# Autodesk Inventor assembly: ASSY_TREBUCHET_DESIGN2
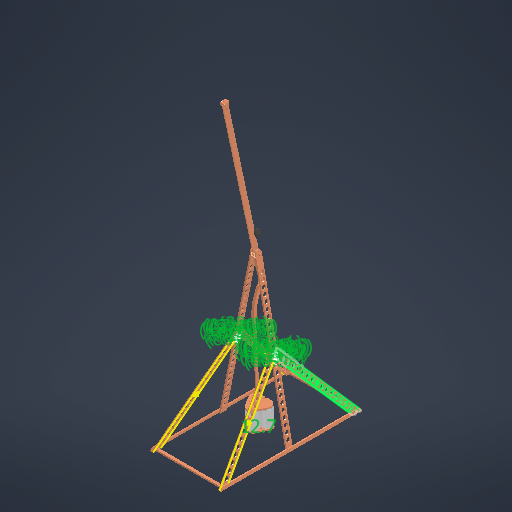
[picture p0: Inventor's stored thumbnail of the model, 512x512]
Saved by Autodesk Inventor 2026.2 (Build 302298010, 298A)
## iProperties
Created: 2026-02-10
Part Number: ASSY_TREBUCHET_DESIGN2
Document SubType Name: Assembly
Designer: 4aida
Mass: 1736.51 g
Surface Area: 8151.09 cm^2
Volume: 2284.88 cm^3
Density: 0.76 g/cm^3
Author: 4aida
## Documents named in this file (17)
- C:\Users\4aida\OneDrive\Documents\GitHub\Design_II_Group6\Trebuchet\WIPPER_TREBUCHET\ASSY_TREBUCHET_DESIGN2.iam
- C:\Users\4aida\OneDrive\Documents\GitHub\Design_II_Group6\Trebuchet\Canette-355ml.ipt
- C:\Users\4aida\OneDrive\Documents\GitHub\Design_II_Group6\Trebuchet\Yellow_dot_squash_ball,Trebuchet.ipt
- C:\Users\4aida\OneDrive\Documents\GitHub\Design_II_Group6\Trebuchet\WIPPER_TREBUCHET\wipper_arm.ipt
- C:\Users\4aida\OneDrive\Documents\GitHub\Design_II_Group6\Trebuchet\COUNTERWEIGHT_OUTSIDE_ARM,TREBUCHET.ipt
- C:\Users\4aida\OneDrive\Documents\GitHub\Design_II_Group6\Trebuchet\WIPPER_TREBUCHET\BASE_FRONT,BACK_TREBUCHET.ipt
- C:\Users\4aida\OneDrive\Documents\GitHub\Design_II_Group6\Trebuchet\WIPPER_TREBUCHET\BASE_SIDEK_TREBUCHET.ipt
- C:\Users\4aida\OneDrive\Documents\GitHub\Design_II_Group6\Trebuchet\WIPPER_TREBUCHET\UPRIGHTS_TREBUCHET.ipt
- C:\Users\4aida\OneDrive\Documents\GitHub\Design_II_Group6\Trebuchet\WIPPER_TREBUCHET\SUPPORTS_TREBUCHET.ipt
- C:\Users\4aida\OneDrive\Documents\GitHub\Design_II_Group6\Trebuchet\WIPPER_TREBUCHET\BOTTOM_PLATE_WEIGHTS_TREBUCHET.ipt
- C:\Users\4aida\OneDrive\Documents\GitHub\Design_II_Group6\Trebuchet\WIPPER_TREBUCHET\TRI_SPACER_TOP_TREBUCHET.ipt
- C:\Users\4aida\OneDrive\Documents\GitHub\Design_II_Group6\Trebuchet\WIPPER_TREBUCHET\MAIN_PIVOT_DOWEL_TREBUCHET.ipt
- C:\Users\4aida\OneDrive\Documents\GitHub\Design_II_Group6\Trebuchet\WIPPER_TREBUCHET\CW_PIVOT_TREBUCHET.ipt
- C:\Users\4aida\OneDrive\Documents\GitHub\Design_II_Group6\Trebuchet\WIPPER_TREBUCHET\TOP_PLATE_WEIGHTS_TREBUCHET.ipt
- C:\Users\4aida\OneDrive\Documents\GitHub\Design_II_Group6\Trebuchet\WIPPER_TREBUCHET\CONTERWEIGHT_SHAFT_TREBUCHET.ipt
- C:\Users\4aida\OneDrive\Documents\GitHub\Design_II_Group6\Trebuchet\WIPPER_TREBUCHET\RELEASE_BLOCK_TREBUCHET.ipt
- C:\Users\4aida\OneDrive\Documents\GitHub\Design_II_Group6\Trebuchet\WIPPER_TREBUCHET\RELEASE_BLOCK_PINS_TREBUCHET.ipt
## Components (27 placed, 16 different names)
1. Yellow_dot_squash_ball,Trebuchet:1 — Mate:45, Mate:85
2. BASE_FRONT,BACK_TREBUCHET:1 — Flush:40, Flush:42, Mate:94
3. BASE_FRONT,BACK_TREBUCHET:3 — Flush:28, Flush:41, Flush:42, Mate:95
4. UPRIGHTS_TREBUCHET:1 — Mate:38, Flush:29, Flush:30, Mate:48, Mate:49, Mate:50, Flush:39, Flush:41, Mate:60, Flush:44, Mate:61, Mate:64, Mate:89, Flush:56, Mate:90, Mate:92
5. UPRIGHTS_TREBUCHET:2 — Flush:31, Flush:32, Mate:46, Mate:47, Mate:50, Flush:39, Angle:1, Flush:40, Mate:58, Mate:59, Flush:43, Mate:88, Flush:54, Mate:91, Mate:93
6. wipper_arm:3 — Mate:39, Mate:44, Mate:45, Mate:55, Mate:56, Flush:45, Mate:66, Mate:75, Mate:76, Mate:77, Mate:78, Mate:79, Mate:82, Mate:85
7. SUPPORTS_TREBUCHET:1 — Flush:30, Mate:49, Mate:92, Mate:94
8. SUPPORTS_TREBUCHET:2 — Flush:32, Mate:46, Flush:53, Mate:91
9. SUPPORTS_TREBUCHET:3 — Flush:29, Mate:48, Flush:55, Mate:90, Mate:95
10. SUPPORTS_TREBUCHET:4 — Flush:31, Mate:47, Mate:93
11. COUNTERWEIGHT_OUTSIDE_ARM,TREBUCHET:3 — Mate:55, Mate:56, Mate:65, Mate:67, Mate:68, Mate:69, Insert:1
12. TRI_SPACER_TOP_TREBUCHET:1 — Mate:60, Flush:44, Mate:61, Mate:76
13. TRI_SPACER_TOP_TREBUCHET:2 — Mate:58, Mate:59, Flush:43, Mate:75
14. MAIN_PIVOT_DOWEL_TREBUCHET:1 — Mate:64, Flush:45
15. CW_PIVOT_TREBUCHET:1 — Mate:65, Mate:66
16. BOTTOM_PLATE_WEIGHTS_TREBUCHET:1 — Flush:48, Flush:49, Mate:74
17. TOP_PLATE_WEIGHTS_TREBUCHET:1 — Mate:67, Mate:68, Mate:69, Mate:70, Mate:71, Mate:72, Mate:73, Flush:48, Flush:49, Mate:74
18. Canette-355ml:4 — Mate:70, Flush:46, Flush:47, Mate:73
19. Canette-355ml:5 — Mate:72, Flush:46
20. Canette-355ml:6 — Mate:71, Flush:47
21. CONTERWEIGHT_SHAFT_TREBUCHET:1 — Insert:1
22. RELEASE_BLOCK_TREBUCHET:1 — Mate:77, Mate:78, Mate:79, Mate:80, Mate:81, Mate:83, Mate:84
23. RELEASE_BLOCK_PINS_TREBUCHET:1 — Mate:80, Flush:50
24. RELEASE_BLOCK_PINS_TREBUCHET:2 — Mate:81, Flush:50, Mate:82
25. RELEASE_BLOCK_PINS_TREBUCHET:3 — Mate:83, Mate:84
26. BASE_SIDEK_TREBUCHET:5 — Mate:88, Flush:53, Flush:54
27. BASE_SIDEK_TREBUCHET:6 — Mate:89, Flush:55, Flush:56
## Relationships (68: Mate 45, Flush 21, Angle 1, Insert 1)
- Flush:28: BASE_FRONT,BACK_TREBUCHET:3
- Mate:38: UPRIGHTS_TREBUCHET:1
- Mate:39: wipper_arm:3
- Mate:44: wipper_arm:3
- Mate:45: Yellow_dot_squash_ball,Trebuchet:1 ↔ wipper_arm:3
- Flush:29: UPRIGHTS_TREBUCHET:1 ↔ SUPPORTS_TREBUCHET:3
- Flush:30: UPRIGHTS_TREBUCHET:1 ↔ SUPPORTS_TREBUCHET:1
- Flush:31: UPRIGHTS_TREBUCHET:2 ↔ SUPPORTS_TREBUCHET:4
- Flush:32: UPRIGHTS_TREBUCHET:2 ↔ SUPPORTS_TREBUCHET:2
- Mate:46: UPRIGHTS_TREBUCHET:2 ↔ SUPPORTS_TREBUCHET:2
- Mate:47: UPRIGHTS_TREBUCHET:2 ↔ SUPPORTS_TREBUCHET:4
- Mate:48: UPRIGHTS_TREBUCHET:1 ↔ SUPPORTS_TREBUCHET:3
- Mate:49: UPRIGHTS_TREBUCHET:1 ↔ SUPPORTS_TREBUCHET:1
- Mate:50: UPRIGHTS_TREBUCHET:1 ↔ UPRIGHTS_TREBUCHET:2
- Flush:39: UPRIGHTS_TREBUCHET:1 ↔ UPRIGHTS_TREBUCHET:2
- Angle:1 (180 deg): UPRIGHTS_TREBUCHET:2
- Flush:40: BASE_FRONT,BACK_TREBUCHET:1 ↔ UPRIGHTS_TREBUCHET:2
- Mate:55: wipper_arm:3 ↔ COUNTERWEIGHT_OUTSIDE_ARM,TREBUCHET:3
- Mate:56: wipper_arm:3 ↔ COUNTERWEIGHT_OUTSIDE_ARM,TREBUCHET:3
- Flush:41: BASE_FRONT,BACK_TREBUCHET:3 ↔ UPRIGHTS_TREBUCHET:1
- Flush:42: BASE_FRONT,BACK_TREBUCHET:1 ↔ BASE_FRONT,BACK_TREBUCHET:3
- Mate:58: UPRIGHTS_TREBUCHET:2 ↔ TRI_SPACER_TOP_TREBUCHET:2
- Mate:59: UPRIGHTS_TREBUCHET:2 ↔ TRI_SPACER_TOP_TREBUCHET:2
- Flush:43: UPRIGHTS_TREBUCHET:2 ↔ TRI_SPACER_TOP_TREBUCHET:2
- Mate:60: UPRIGHTS_TREBUCHET:1 ↔ TRI_SPACER_TOP_TREBUCHET:1
- Flush:44: UPRIGHTS_TREBUCHET:1 ↔ TRI_SPACER_TOP_TREBUCHET:1
- Mate:61: UPRIGHTS_TREBUCHET:1 ↔ TRI_SPACER_TOP_TREBUCHET:1
- Mate:64: UPRIGHTS_TREBUCHET:1 ↔ MAIN_PIVOT_DOWEL_TREBUCHET:1
- Flush:45: wipper_arm:3 ↔ MAIN_PIVOT_DOWEL_TREBUCHET:1
- Mate:65: COUNTERWEIGHT_OUTSIDE_ARM,TREBUCHET:3 ↔ CW_PIVOT_TREBUCHET:1
- Mate:66: wipper_arm:3 ↔ CW_PIVOT_TREBUCHET:1
- Mate:67: COUNTERWEIGHT_OUTSIDE_ARM,TREBUCHET:3 ↔ TOP_PLATE_WEIGHTS_TREBUCHET:1
- Mate:68: COUNTERWEIGHT_OUTSIDE_ARM,TREBUCHET:3 ↔ TOP_PLATE_WEIGHTS_TREBUCHET:1
- Mate:69: COUNTERWEIGHT_OUTSIDE_ARM,TREBUCHET:3 ↔ TOP_PLATE_WEIGHTS_TREBUCHET:1
- Mate:70: TOP_PLATE_WEIGHTS_TREBUCHET:1 ↔ Canette-355ml:4
- Mate:71: TOP_PLATE_WEIGHTS_TREBUCHET:1 ↔ Canette-355ml:6
- Mate:72: TOP_PLATE_WEIGHTS_TREBUCHET:1 ↔ Canette-355ml:5
- Flush:46: Canette-355ml:4 ↔ Canette-355ml:5
- Flush:47: Canette-355ml:4 ↔ Canette-355ml:6
- Mate:73: TOP_PLATE_WEIGHTS_TREBUCHET:1 ↔ Canette-355ml:4
- Flush:48: BOTTOM_PLATE_WEIGHTS_TREBUCHET:1 ↔ TOP_PLATE_WEIGHTS_TREBUCHET:1
- Flush:49: BOTTOM_PLATE_WEIGHTS_TREBUCHET:1 ↔ TOP_PLATE_WEIGHTS_TREBUCHET:1
- Mate:74 (112 mm): BOTTOM_PLATE_WEIGHTS_TREBUCHET:1 ↔ TOP_PLATE_WEIGHTS_TREBUCHET:1
- Mate:75: wipper_arm:3 ↔ TRI_SPACER_TOP_TREBUCHET:2
- Mate:76: wipper_arm:3 ↔ TRI_SPACER_TOP_TREBUCHET:1
- Insert:1: COUNTERWEIGHT_OUTSIDE_ARM,TREBUCHET:3 ↔ CONTERWEIGHT_SHAFT_TREBUCHET:1
- Mate:77: wipper_arm:3 ↔ RELEASE_BLOCK_TREBUCHET:1
- Mate:78: wipper_arm:3 ↔ RELEASE_BLOCK_TREBUCHET:1
- Mate:79: wipper_arm:3 ↔ RELEASE_BLOCK_TREBUCHET:1
- Mate:80: RELEASE_BLOCK_TREBUCHET:1 ↔ RELEASE_BLOCK_PINS_TREBUCHET:1
- Mate:81: RELEASE_BLOCK_TREBUCHET:1 ↔ RELEASE_BLOCK_PINS_TREBUCHET:2
- Flush:50: RELEASE_BLOCK_PINS_TREBUCHET:1 ↔ RELEASE_BLOCK_PINS_TREBUCHET:2
- Mate:82: wipper_arm:3 ↔ RELEASE_BLOCK_PINS_TREBUCHET:2
- Mate:83: RELEASE_BLOCK_TREBUCHET:1 ↔ RELEASE_BLOCK_PINS_TREBUCHET:3
- Mate:84 (10 mm): RELEASE_BLOCK_TREBUCHET:1 ↔ RELEASE_BLOCK_PINS_TREBUCHET:3
- Mate:85: Yellow_dot_squash_ball,Trebuchet:1 ↔ wipper_arm:3
- Mate:88: UPRIGHTS_TREBUCHET:2 ↔ BASE_SIDEK_TREBUCHET:5
- Flush:53: SUPPORTS_TREBUCHET:2 ↔ BASE_SIDEK_TREBUCHET:5
- Flush:54: UPRIGHTS_TREBUCHET:2 ↔ BASE_SIDEK_TREBUCHET:5
- Mate:89: UPRIGHTS_TREBUCHET:1 ↔ BASE_SIDEK_TREBUCHET:6
- Flush:55: SUPPORTS_TREBUCHET:3 ↔ BASE_SIDEK_TREBUCHET:6
- Flush:56: UPRIGHTS_TREBUCHET:1 ↔ BASE_SIDEK_TREBUCHET:6
- Mate:90: UPRIGHTS_TREBUCHET:1 ↔ SUPPORTS_TREBUCHET:3
- Mate:91: UPRIGHTS_TREBUCHET:2 ↔ SUPPORTS_TREBUCHET:2
- Mate:92: UPRIGHTS_TREBUCHET:1 ↔ SUPPORTS_TREBUCHET:1
- Mate:93: UPRIGHTS_TREBUCHET:2 ↔ SUPPORTS_TREBUCHET:4
- Mate:94: BASE_FRONT,BACK_TREBUCHET:1 ↔ SUPPORTS_TREBUCHET:1
- Mate:95: BASE_FRONT,BACK_TREBUCHET:3 ↔ SUPPORTS_TREBUCHET:3
